# Autodesk Inventor assembly: ElbowAssembly
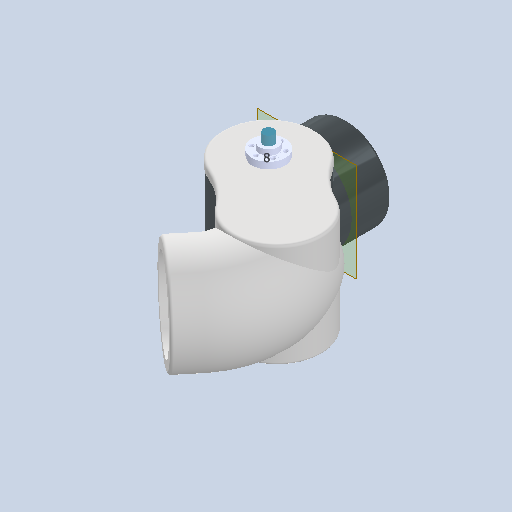
[picture p0: Inventor's stored thumbnail of the model, 512x512]
Saved by Autodesk Inventor 2024 (Build 280153000, 153)
## iProperties
Created: 2024-03-12
Part Number: ElbowAssembly
Document SubType Name: Assembly
Designer: Irwin
Author: Irwin
## Documents named in this file (7)
- C:\Users\anyangoe\Desktop\WholeRobot\ElbowAssembly.iam
- C:\Users\anyangoe\Desktop\WholeRobot\ElbowIn.ipt
- C:\Users\anyangoe\Desktop\WholeRobot\ElbowOut.ipt
- C:\Users\anyangoe\Desktop\WholeRobot\8mmShaft.ipt
- C:\Users\anyangoe\Desktop\WholeRobot\mounting-hub-8mm-shaft-m3-holes.ipt
- C:\Users\anyangoe\Desktop\WholeRobot\GT2 Timing Pulley 20T 10mm - Bore_8mm.iam
- C:\Users\anyangoe\Desktop\WholeRobot\FlangedBearing.ipt
## Components (8 placed, 6 different names)
1. ElbowIn:1 — Mate:1, Mate:2, Mate:3, Mate:4, Mate:11, Mate:14, Mate:15
2. ElbowOut:1 — Mate:3, Mate:4, Mate:5, Flush:1, Mate:8, Mate:9
3. 8mmShaft:1 — Mate:5, Flush:1, Mate:6, Mate:7, Mate:10, Mate:12, Mate:13
4. mounting-hub-8mm-shaft-m3-holes:1 — Mate:6, Mate:9
5. mounting-hub-8mm-shaft-m3-holes:2 — Mate:7, Mate:8
6. GT2 Timing Pulley 20T 10mm - Bore_8mm:1 [sub-assembly] — Mate:10, Mate:11
7. FlangedBearing:1 — Mate:13, Mate:15
8. FlangedBearing:2 — Mate:12, Mate:14
## Relationships (16: Mate 15, Flush 1)
- Mate:1: ElbowIn:1
- Mate:2: ElbowIn:1
- Mate:3: ElbowIn:1 ↔ ElbowOut:1
- Mate:4 (2 mm): ElbowIn:1 ↔ ElbowOut:1
- Mate:5: ElbowOut:1 ↔ 8mmShaft:1
- Flush:1 (-15 mm): ElbowOut:1 ↔ 8mmShaft:1
- Mate:6: 8mmShaft:1 ↔ mounting-hub-8mm-shaft-m3-holes:1
- Mate:7: 8mmShaft:1 ↔ mounting-hub-8mm-shaft-m3-holes:2
- Mate:8: ElbowOut:1 ↔ mounting-hub-8mm-shaft-m3-holes:2
- Mate:9: ElbowOut:1 ↔ mounting-hub-8mm-shaft-m3-holes:1
- Mate:10: 8mmShaft:1 ↔ GT2 Timing Pulley 20T 10mm - Bore_8mm:1
- Mate:11 (20 mm): ElbowIn:1 ↔ GT2 Timing Pulley 20T 10mm - Bore_8mm:1
- Mate:12: 8mmShaft:1 ↔ FlangedBearing:2
- Mate:13: 8mmShaft:1 ↔ FlangedBearing:1
- Mate:14: ElbowIn:1 ↔ FlangedBearing:2
- Mate:15: ElbowIn:1 ↔ FlangedBearing:1
